# Autodesk Inventor assembly: 4mmShaftSeal
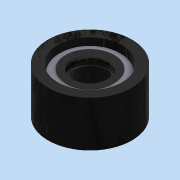
[picture p0: Inventor's stored thumbnail of the model, 180x180]
Saved by Autodesk Inventor 2017 (Build 210142000, 142)
## iProperties
Created: 2016-10-13
Part Number: 4mmShaftSeal
Document SubType Name: Assembly
Designer: techn
Author: techn
## Documents named in this file (3)
- D:\OneDrive\Documents\Other Projects\Submarine\CAD\aft\ShaftSeal\4mmShaftSeal.iam
- D:\OneDrive\Documents\Other Projects\Submarine\CAD\aft\ShaftSeal\CoilSpring.ipt
- D:\OneDrive\Documents\Other Projects\Submarine\CAD\aft\ShaftSeal\RubberMould.ipt
## Components (2 placed, 2 different names)
1. CoilSpring:1 — Mate:1, Rigid:1
2. RubberMould:1 — Mate:1, Rigid:1
## Relationships (2: Mate 1, WeldJoint 1)
- Mate:1: CoilSpring:1 ↔ RubberMould:1
- Rigid:1 [WeldJoint]: CoilSpring:1 ↔ RubberMould:1
